# Autodesk Inventor assembly: Assembly1
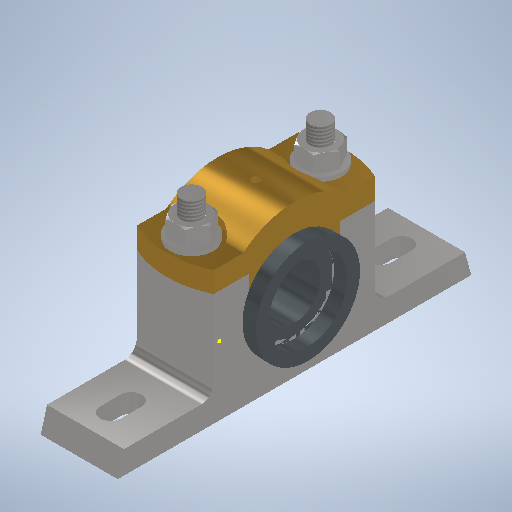
[picture p0: Inventor's stored thumbnail of the model, 512x512]
Saved by Autodesk Inventor 2025.2 (Build 292293000, 293)
## iProperties
Created: 2025-04-15
Part Number: Assembly1
Document SubType Name: Assembly
Designer: bless
Author: bless
## Documents named in this file (8)
- C:\Users\bless\OneDrive - Conestoga College\Documents\Inventor\8071W25\final evaluation 9005538\FINAL EXAM\Assembly1.iam
- C:\Users\bless\OneDrive - Conestoga College\Documents\Inventor\8071W25\final evaluation 9005538\cap.ipt
- C:\Users\bless\OneDrive - Conestoga College\Documents\Inventor\8071W25\final evaluation 9005538\base.ipt
- C:\Users\bless\OneDrive - Conestoga College\Documents\Inventor\8071W25\final evaluation 9005538\BEARING TOP.ipt
- C:\Users\bless\OneDrive - Conestoga College\Documents\Inventor\8071W25\final evaluation 9005538\BEARING BOTTOM.ipt
- C:\Users\bless\OneDrive - Conestoga College\Documents\Inventor\8071W25\final evaluation 9005538\SCREW.ipt
- C:\Users\bless\OneDrive - Conestoga College\Documents\Inventor\Content Center Files\R2025\en-US\AS 1237 (D1)\AS 1237 - 10 mm(5).ipt
- C:\Users\bless\OneDrive - Conestoga College\Documents\Inventor\Content Center Files\R2025\en-US\AS 1112 (2)\AS 1112 - M10  Type 5.ipt
## Components (9 placed, 7 different names)
1. cap:1 — Flush:1, Flush:2, Insert:1, Insert:2
2. base:1 — Flush:1, Flush:3, Flush:4, Flush:5, Flush:6, Flush:7, Flush:8, Flush:9, Flush:10
3. BEARING TOP:1 — Flush:2, Flush:3, Flush:4
4. BEARING BOTTOM:1 — Flush:5, Flush:6, Flush:7, Flush:8
5. SCREW:1 — Flush:9, Flush:10
6. AS 1237 (D1) 10 mm:1 — Insert:1, Insert:3
7. AS 1237 (D1) 10 mm:2 — Insert:2, Insert:4
8. AS 1112 (2) - Metric M10  Type 5:1 — Insert:3
9. AS 1112 (2) - Metric M10  Type 5:2 — Insert:4
## Relationships (14: Flush 10, Insert 4)
- Flush:1: cap:1 ↔ base:1
- Flush:2: cap:1 ↔ BEARING TOP:1
- Flush:3: base:1 ↔ BEARING TOP:1
- Flush:4: base:1 ↔ BEARING TOP:1
- Flush:5: base:1 ↔ BEARING BOTTOM:1
- Flush:6: base:1 ↔ BEARING BOTTOM:1
- Flush:7: base:1 ↔ BEARING BOTTOM:1
- Flush:8: base:1 ↔ BEARING BOTTOM:1
- Flush:9: base:1 ↔ SCREW:1
- Flush:10: base:1 ↔ SCREW:1
- Insert:1: cap:1 ↔ AS 1237 (D1) 10 mm:1
- Insert:2: cap:1 ↔ AS 1237 (D1) 10 mm:2
- Insert:3: AS 1237 (D1) 10 mm:1 ↔ AS 1112 (2) - Metric M10  Type 5:1
- Insert:4: AS 1237 (D1) 10 mm:2 ↔ AS 1112 (2) - Metric M10  Type 5:2
